# Autodesk Inventor assembly: linear slide
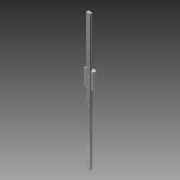
[picture p0: Inventor's stored thumbnail of the model, 180x180]
Saved by Autodesk Inventor 2015 SP1 (Build 190203100, 203)
## iProperties
Created: 2015-02-03
Part Number: linear slide
Document SubType Name: Assembly
Designer: Joseph
Author: Joseph
## Documents named in this file (3)
- C:\Users\Joseph\Documents\GitHub\mchp_kossel\Printer\linear slide.iam
- C:\Users\Joseph\Documents\GitHub\mchp_kossel\Printer\slide.ipt
- C:\Users\Joseph\Documents\GitHub\mchp_kossel\Printer\slide rail.ipt
## Components (2 placed, 2 different names)
1. slide:1 — Mate:1, Mate:2
2. slide rail:1 — Mate:1, Mate:2
## Relationships (2: Mate 2)
- Mate:1: slide:1 ↔ slide rail:1
- Mate:2: slide:1 ↔ slide rail:1
